# Autodesk Inventor assembly: 知能ロボコン発射筒1.1
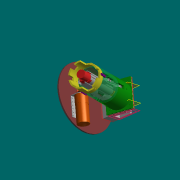
[picture p0: Inventor's stored thumbnail of the model, 180x180]
Saved by Autodesk Inventor 2013 (Build 170138000, 138)
## iProperties
Created: 2014-05-31
Part Number: 知能ロボコン発射筒1.1
Document SubType Name: Assembly
Designer: horumo136
Author: horumo136
## Documents named in this file (14)
- C:\Users\horumo136\Documents\知能ロボコン発射筒1.1.iam
- C:\Users\horumo136\Documents\知能ロボコン外筒改1.1.ipt
- C:\Users\horumo136\Documents\知能ロボコン外筒改1.2.ipt
- C:\Users\horumo136\Documents\知能ロボコンショウレックス戸草.ipt
- C:\Users\horumo136\Documents\知能ロボコンラックギア.ipt
- C:\Users\horumo136\Documents\知能ロボコンシリンダ２.ipt
- C:\Users\horumo136\Documents\知能ロボコンばね112038.ipt
- C:\Users\horumo136\Documents\知能ロボコンばね受け.iam
- C:\Users\horumo136\Documents\知能ロボコン発射口.ipt
- C:\Users\horumo136\Documents\知能ロボコンシリンダ延長.ipt
- C:\Users\horumo136\Documents\知能ロボコン540gia.iam
- C:\Users\horumo136\Documents\知能ロボコン砲身止め.ipt
- C:\Users\horumo136\Documents\知能ロボコン土台1.1.ipt
- C:\Users\horumo136\Documents\知能ロボコンターンテーブル1.1.ipt
## Components (20 placed, 13 different names)
1. 知能ロボコン外筒改1.1:1 — メイト:1, メイト:2, メイト:3, メイト:4, メイト:6, メイト:84, メイト:85, メイト:86, メイト:87
2. 知能ロボコン外筒改1.2:1 — メイト:1, メイト:2, メイト:3, メイト:5, メイト:7, メイト:8, メイト:9, メイト:35, メイト:36, メイト:37, メイト:50, メイト:59, メイト:60, メイト:62, メイト:63, メイト:65, メイト:66
3. 知能ロボコンラックギア:1 — メイト:26, メイト:27, メイト:28
4. 知能ロボコンシリンダ２:1 — メイト:16, メイト:26, メイト:27, メイト:28, メイト:38, メイト:39, メイト:51, メイト:52
5. 知能ロボコンばね112038:1 — メイト:13, メイト:14, メイト:15, メイト:68
6. 知能ロボコンばね受け:1 [sub-assembly] — メイト:13, メイト:14, メイト:15, メイト:16, メイト:68, メイト:81, メイト:82, メイト:83, メイト:84, メイト:85, メイト:86, メイト:87
7. 知能ロボコン発射口:1 — メイト:35, メイト:36, メイト:37, メイト:50, メイト:61, メイト:64, メイト:67
8. 知能ロボコンシリンダ延長:1 — メイト:38, メイト:39, メイト:51, メイト:52
9. 知能ロボコン540gia:1 [sub-assembly] — メイト:94, メイト:95, メイト:96
10. 知能ロボコン砲身止め:1 — メイト:59, メイト:60, メイト:61
11. 知能ロボコン砲身止め:2 — メイト:62, メイト:63, メイト:64
12. 知能ロボコン砲身止め:3 — メイト:65, メイト:66, メイト:67
13. 知能ロボコン土台1.1:1 — メイト:81, メイト:82, メイト:83
14. 知能ロボコンターンテーブル1.1:1 — メイト:94, メイト:95, メイト:96
15. 知能ロボコンショウレックス戸草:6 — メイト:4, メイト:5, メイト:6
16. 知能ロボコンショウレックス戸草:7
17. 知能ロボコンショウレックス戸草:8
18. 知能ロボコンショウレックス戸草:2 — メイト:7, メイト:8, メイト:9
19. 知能ロボコンショウレックス戸草:9
20. 知能ロボコンショウレックス戸草:10
## Component patterns: (3 elements, first: 知能ロボコンショウレックス戸草:6), (3 elements, first: 知能ロボコンショウレックス戸草:2)
## Relationships (44: Mate 44)
- メイト:1 [Mate]: 知能ロボコン外筒改1.1:1 ↔ 知能ロボコン外筒改1.2:1
- メイト:2 [Mate]: 知能ロボコン外筒改1.1:1 ↔ 知能ロボコン外筒改1.2:1
- メイト:3 [Mate]: 知能ロボコン外筒改1.1:1 ↔ 知能ロボコン外筒改1.2:1
- メイト:4 [Mate]: 知能ロボコン外筒改1.1:1 ↔ 知能ロボコンショウレックス戸草:6
- メイト:5 [Mate]: 知能ロボコン外筒改1.2:1 ↔ 知能ロボコンショウレックス戸草:6
- メイト:6 [Mate]: 知能ロボコン外筒改1.1:1 ↔ 知能ロボコンショウレックス戸草:6
- メイト:7 [Mate]: 知能ロボコン外筒改1.2:1 ↔ 知能ロボコンショウレックス戸草:2
- メイト:8 [Mate]: 知能ロボコン外筒改1.2:1 ↔ 知能ロボコンショウレックス戸草:2
- メイト:9 [Mate]: 知能ロボコン外筒改1.2:1 ↔ 知能ロボコンショウレックス戸草:2
- メイト:13 [Mate]: 知能ロボコンばね112038:1 ↔ 知能ロボコンばね受け:1
- メイト:14 [Mate]: 知能ロボコンばね112038:1 ↔ 知能ロボコンばね受け:1
- メイト:15 [Mate]: 知能ロボコンばね112038:1 ↔ 知能ロボコンばね受け:1
- メイト:16 [Mate]: 知能ロボコンシリンダ２:1 ↔ 知能ロボコンばね受け:1
- メイト:26 [Mate]: 知能ロボコンラックギア:1 ↔ 知能ロボコンシリンダ２:1
- メイト:27 [Mate]: 知能ロボコンラックギア:1 ↔ 知能ロボコンシリンダ２:1
- メイト:28 [Mate]: 知能ロボコンラックギア:1 ↔ 知能ロボコンシリンダ２:1
- メイト:35 [Mate]: 知能ロボコン外筒改1.2:1 ↔ 知能ロボコン発射口:1
- メイト:36 [Mate]: 知能ロボコン外筒改1.2:1 ↔ 知能ロボコン発射口:1
- メイト:37 [Mate]: 知能ロボコン外筒改1.2:1 ↔ 知能ロボコン発射口:1
- メイト:38 [Mate]: 知能ロボコンシリンダ２:1 ↔ 知能ロボコンシリンダ延長:1
- メイト:39 [Mate]: 知能ロボコンシリンダ２:1 ↔ 知能ロボコンシリンダ延長:1
- メイト:50 [Mate]: 知能ロボコン外筒改1.2:1 ↔ 知能ロボコン発射口:1
- メイト:51 [Mate]: 知能ロボコンシリンダ２:1 ↔ 知能ロボコンシリンダ延長:1
- メイト:52 [Mate]: 知能ロボコンシリンダ２:1 ↔ 知能ロボコンシリンダ延長:1
- メイト:59 [Mate]: 知能ロボコン外筒改1.2:1 ↔ 知能ロボコン砲身止め:1
- メイト:60 [Mate]: 知能ロボコン外筒改1.2:1 ↔ 知能ロボコン砲身止め:1
- メイト:61 [Mate]: 知能ロボコン発射口:1 ↔ 知能ロボコン砲身止め:1
- メイト:62 [Mate]: 知能ロボコン外筒改1.2:1 ↔ 知能ロボコン砲身止め:2
- メイト:63 [Mate]: 知能ロボコン外筒改1.2:1 ↔ 知能ロボコン砲身止め:2
- メイト:64 [Mate]: 知能ロボコン発射口:1 ↔ 知能ロボコン砲身止め:2
- メイト:65 [Mate]: 知能ロボコン外筒改1.2:1 ↔ 知能ロボコン砲身止め:3
- メイト:66 [Mate]: 知能ロボコン外筒改1.2:1 ↔ 知能ロボコン砲身止め:3
- メイト:67 [Mate]: 知能ロボコン発射口:1 ↔ 知能ロボコン砲身止め:3
- メイト:68 [Mate]: 知能ロボコンばね112038:1 ↔ 知能ロボコンばね受け:1
- メイト:81 [Mate]: 知能ロボコンばね受け:1 ↔ 知能ロボコン土台1.1:1
- メイト:82 [Mate]: 知能ロボコンばね受け:1 ↔ 知能ロボコン土台1.1:1
- メイト:83 [Mate]: 知能ロボコンばね受け:1 ↔ 知能ロボコン土台1.1:1
- メイト:84 [Mate]: 知能ロボコン外筒改1.1:1 ↔ 知能ロボコンばね受け:1
- メイト:85 [Mate]: 知能ロボコン外筒改1.1:1 ↔ 知能ロボコンばね受け:1
- メイト:86 [Mate]: 知能ロボコン外筒改1.1:1 ↔ 知能ロボコンばね受け:1
- メイト:87 [Mate]: 知能ロボコン外筒改1.1:1 ↔ 知能ロボコンばね受け:1
- メイト:94 [Mate]: 知能ロボコン540gia:1 ↔ 知能ロボコンターンテーブル1.1:1
- メイト:95 [Mate]: 知能ロボコン540gia:1 ↔ 知能ロボコンターンテーブル1.1:1
- メイト:96 [Mate]: 知能ロボコン540gia:1 ↔ 知能ロボコンターンテーブル1.1:1
